# Autodesk Inventor assembly: assyEscapement
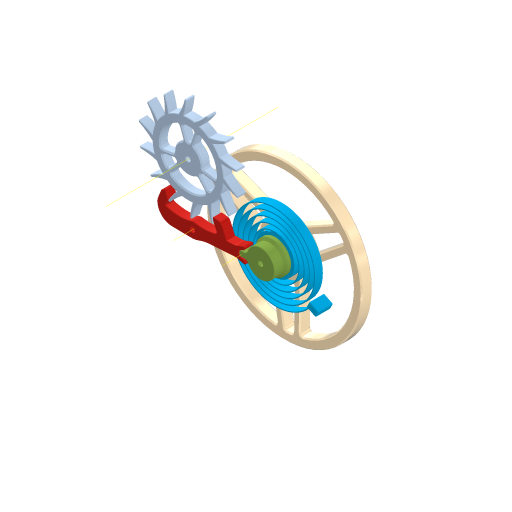
[picture p0: Inventor's stored thumbnail of the model, 512x512]
Saved by Autodesk Inventor 2023 (Build 270158000, 158)
## iProperties
Created: 2023-02-14
Part Number: assyEscapement
Document SubType Name: Assembly
Designer: Aditya
Author: Aditya
## Documents named in this file (3)
- C:\Users\Aditya\Documents\Inventor\Tourbillon\assyEscapement.iam
- C:\Users\Aditya\Documents\Inventor\Tourbillon\escapement.ipt
- C:\Users\Aditya\Documents\Inventor\Tourbillon\balanceWheel.ipt
## Components (2 placed, 2 different names)
1. escapement:1 — Flush:1, Flush:2, Flush:3, Mate:1, Flush:4, Mate:2
2. balanceWheel:1 — Mate:1, Flush:4, Angle:1, Mate:2
## Relationships (7: Flush 4, Mate 2, Angle 1)
- Flush:1: escapement:1
- Flush:2: escapement:1
- Flush:3: escapement:1
- Mate:1: escapement:1 ↔ balanceWheel:1
- Flush:4: escapement:1 ↔ balanceWheel:1
- Angle:1 (28 deg): balanceWheel:1
- Mate:2: escapement:1 ↔ balanceWheel:1
